# Autodesk Inventor assembly: Field Crater Left Mineral
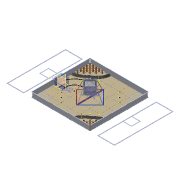
[picture p0: Inventor's stored thumbnail of the model, 180x180]
Saved by Autodesk Inventor 2018 (Build 220112000, 112)
## iProperties
Created: 2018-08-21
Part Number: Field Crater Left Mineral
Description: STEP AP214
Document SubType Name: Assembly
Designer: ball
Sending System: SolidWorks 2018
Preprocessor: SwSTEP 2.0
Title: Production Full Field 0-2 Final Final.STEP
Revision Number: ANY
## Documents named in this file (12)
- C:\FTC\FTC8863CAD\2018Robot\Field\Field Crater Left Mineral.iam
- C:\FTC\FTC8863CAD\2018Robot\Field\Perimeter and Tiles.iam
- C:\FTC\FTC8863CAD\2018Robot\Field\Corner Crater Rim.iam
- C:\FTC\FTC8863CAD\2018Robot\Field\Player Station.ipt
- C:\FTC\FTC8863CAD\2018Robot\Field\Production Lander.iam
- C:\FTC\FTC8863CAD\2018Robot\Field\Center Diamond.ipt
- C:\FTC\FTC8863CAD\2018Robot\Field\1 tile safe zone.ipt
- C:\FTC\FTC8863CAD\2018Robot\Field\Sample Field.ipt
- C:\FTC\FTC8863CAD\2018Robot\Field\Game Piece Array.iam
- C:\FTC\FTC8863CAD\2018Robot\Field\Target in sleeve.ipt
- C:\FTC\FTC8863CAD\2018Robot\Field\robot.ipt
- C:\FTC\FTC8863CAD\2018Robot\Field\am-2850 wiffle base Ball.ipt
## Components (24 placed, 23 different names)
1. Perimeter and Tiles_1 [sub-assembly] — Mate:1, Mate:3, Mate:4
2. Corner Crater Rim_2 [sub-assembly]
3. Corner Crater Rim_3 [sub-assembly]
4. Player Station_4
5. Player Station_5
6. Production Lander_6 [sub-assembly] — Angle:1, Mate:2, Flush:1
7. Center Diamond_7
8. 1 tile safe zone_8
9. 1 tile safe zone_9
10. Sample Field_10 — Mate:5
11. Sample Field_11
12. Sample Field_12
13. Sample Field_13
14. 1 tile safe zone_14
15. 1 tile safe zone_15
16. Game Piece Array_16 [sub-assembly]
17. Game Piece Array_17 [sub-assembly]
18. Target in sleeve_18
19. Target in sleeve_19
20. Target in sleeve_20
21. Target in sleeve_21
22. robot:1 — Mate:1, Angle:1, Mate:2, Flush:1
23. robot:2 — Mate:3, Mate:4
24. am-2850 wiffle base Ball:1 — Mate:5
## Relationships (7: Mate 5, Angle 1, Flush 1)
- Mate:1: Perimeter and Tiles_1 ↔ robot:1
- Angle:1 (0 deg): Production Lander_6 ↔ robot:1
- Mate:2 (12.7 mm): Production Lander_6 ↔ robot:1
- Flush:1: Production Lander_6 ↔ robot:1
- Mate:3: Perimeter and Tiles_1 ↔ robot:2
- Mate:4 (50.8 mm): Perimeter and Tiles_1 ↔ robot:2
- Mate:5: Sample Field_10 ↔ am-2850 wiffle base Ball:1
